# Autodesk Inventor assembly: O's ASSEMBLY
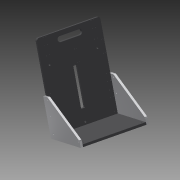
[picture p0: Inventor's stored thumbnail of the model, 180x180]
Saved by Autodesk Inventor 2014 (Build 180170000, 170)
## iProperties
Created: 2013-12-17
Part Number: O's ASSEMBLY
Document SubType Name: Assembly
Designer: orlando
Author: orlando
## Documents named in this file (5)
- \\GRISTLE\speco\GitHub\ConceptFORGE\Wally\O's ASSEMBLY.iam
- \\GRISTLE\speco\GitHub\ConceptFORGE\Wally\bottom.ipt
- \\GRISTLE\speco\GitHub\ConceptFORGE\Wally\side support.ipt
- \\GRISTLE\speco\GitHub\ConceptFORGE\Wally\side support1.ipt
- \\GRISTLE\speco\GitHub\ConceptFORGE\Wally\O'S BACK BOARD.ipt
## Components (4 placed, 4 different names)
1. O'S BACK BOARD:1 — Mate:9, Mate:10, Mate:13
2. bottom:1 — Mate:11, Mate:12, Mate:13
3. side support:1 — Mate:9, Mate:12
4. side support1:1 — Mate:10, Mate:11
## Relationships (5: Mate 5)
- Mate:9: O'S BACK BOARD:1 ↔ side support:1
- Mate:10: O'S BACK BOARD:1 ↔ side support1:1
- Mate:11: bottom:1 ↔ side support1:1
- Mate:12: bottom:1 ↔ side support:1
- Mate:13: O'S BACK BOARD:1 ↔ bottom:1
